# Autodesk Inventor assembly: collector wheel mounted on low channel
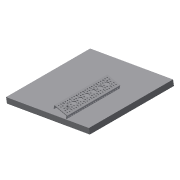
[picture p0: Inventor's stored thumbnail of the model, 180x180]
Saved by Autodesk Inventor 2018 (Build 220112000, 112)
## iProperties
Created: 2019-02-06
Part Number: collector wheel mounted on low channel
Document SubType Name: Assembly
Designer: ball
Author: ball
## Documents named in this file (4)
- C:\FTC\FTC8863CAD\2018Robot\collector wheel mounted on low channel.iam
- C:\FTC\FTC8863CAD\GoBilda\1121 Parts\1121-0007-0192.ipt
- C:\FTC\FTC8863CAD\2018Robot\Floor.ipt
- C:\FTC\FTC8863CAD\GoBilda\1601 Parts\1601-0014-0006.ipt
## Components (3 placed, 3 different names)
1. 1121-0007-0192:1 — Mate:1, Flush:1, Angle:1, Mate:6, Mate:7
2. Floor:1 — Mate:1, Flush:1, Angle:1
3. 1601-0014-0006:1 — Mate:6, Mate:7
## Relationships (5: Mate 3, Flush 1, Angle 1)
- Mate:1 (2.032 mm): 1121-0007-0192:1 ↔ Floor:1
- Flush:1: 1121-0007-0192:1 ↔ Floor:1
- Angle:1 (158 deg): 1121-0007-0192:1 ↔ Floor:1
- Mate:6: 1121-0007-0192:1 ↔ 1601-0014-0006:1
- Mate:7: 1121-0007-0192:1 ↔ 1601-0014-0006:1
